# Autodesk Inventor assembly: charge_assem
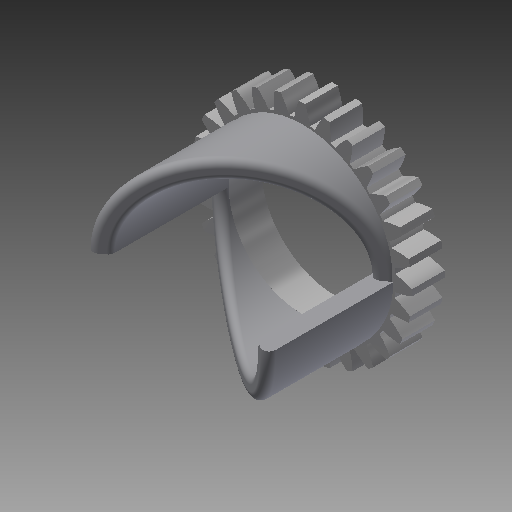
[picture p0: Inventor's stored thumbnail of the model, 512x512]
Saved by Autodesk Inventor 2018 (Build 220112000, 112)
## iProperties
Created: 2018-02-07
Part Number: charge_assem
Material: Générique
Document SubType Name: Assembly
Designer: Mephiro
Author: Mephiro
## Documents named in this file (3)
- C:\Users\Mephiro\Google Drive\Robot_cup_3D\Canon_v3\charge_assem.iam
- C:\Users\Mephiro\Google Drive\Robot_cup_3D\Canon_v3\Canon_assem\Design Accelerator\Engrenage cylindrique11.ipt
- C:\Users\Mephiro\Google Drive\Robot_cup_3D\Canon_v3\charge.ipt
## Components (2 placed, 2 different names)
1. Engrenage cylindrique1:1 — Placage:1, Placage:2
2. charge:1 — Placage:1, Placage:2
## Relationships (2: Mate 2)
- Placage:1 [Mate]: Engrenage cylindrique1:1 ↔ charge:1
- Placage:2 [Mate]: Engrenage cylindrique1:1 ↔ charge:1
